# Autodesk Inventor assembly: Linear slides
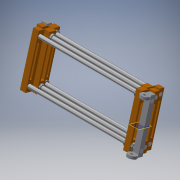
[picture p0: Inventor's stored thumbnail of the model, 180x180]
Saved by Autodesk Inventor 2019 (Build 230136000, 136)
## iProperties
Created: 2019-03-07
Part Number: Linear slides
Document SubType Name: Assembly
Designer: Delta
Mass: 697.362 g
Surface Area: 1389.66 cm^2
Volume: 258.282 cm^3
Density: 2.7 g/cm^3
Author: Delta
## Documents named in this file (6)
- C:\Robotics\2019-20_CAD\Linear Slides\Linear slides.iam
- C:\Robotics\2019-20_CAD\Linear Slides\Block_3-8.ipt
- C:\Robotics\2019-20_CAD\Linear Slides\rod_3-8_12 inch.ipt
- C:\Robotics\COTSParts\Bearings - McMaster\60595K120_FIXED ALIGNMENT  LINEAR BALL BRNG.ipt
- C:\Robotics\2019-20_CAD\Linear Slides\axil mount.ipt
- C:\Robotics\2019-20_CAD\Linear Slides\end piece.ipt
## Components (20 placed, 5 different names)
1. Block_3-8:1 — Mate:3, Mate:4, Mate:9, Mate:11, Mate:13, Mate:14, Mate:20
2. Block_3-8:2 — Mate:5, Mate:6, Mate:10, Mate:12, Mate:17, Mate:18, Mate:23, Mate:24
3. rod_3-8_12 inch:1 — Mate:4, Mate:11, Mate:27, Flush:7, Mate:49
4. rod_3-8_12 inch:2 — Mate:5, Mate:10, Flush:4, Mate:31
5. rod_3-8_12 inch:3 — Mate:3, Mate:9, Mate:28, Mate:50
6. rod_3-8_12 inch:4 — Mate:6, Mate:12, Flush:4, Mate:32, Flush:5
7. rod_3-8_12 inch:5 — Mate:25, Flush:2, Mate:30, Mate:43
8. rod_3-8_12 inch:6 — Mate:26, Mate:29, Flush:3, Flush:6, Mate:44
9. 60595K120_FIXED ALIGNMENT  LINEAR BALL BRNG:2 — Mate:13, Mate:26, Flush:1
10. 60595K120_FIXED ALIGNMENT  LINEAR BALL BRNG:4 — Mate:14, Mate:20, Mate:25, Flush:1
11. 60595K120_FIXED ALIGNMENT  LINEAR BALL BRNG:5 — Mate:17, Mate:23, Mate:28
12. 60595K120_FIXED ALIGNMENT  LINEAR BALL BRNG:6 — Mate:18, Mate:24, Mate:27
13. axil mount:1 — Mate:29, Flush:2, Flush:3, Mate:30
14. end piece:1 — Mate:31, Mate:32, Flush:5
15. Block_3-8:3 — Flush:6, Mate:43, Mate:44, Mate:45, Mate:46, Mate:47, Mate:48
16. Block_3-8:4 — Mate:39, Mate:40, Mate:41, Mate:42, Flush:7, Mate:49, Mate:50
17. 60595K120_FIXED ALIGNMENT  LINEAR BALL BRNG:7 — Mate:45, Mate:46
18. 60595K120_FIXED ALIGNMENT  LINEAR BALL BRNG:8 — Mate:47, Mate:48
19. 60595K120_FIXED ALIGNMENT  LINEAR BALL BRNG:9 — Mate:39, Mate:40
20. 60595K120_FIXED ALIGNMENT  LINEAR BALL BRNG:10 — Mate:41, Mate:42
## Relationships (42: Mate 35, Flush 7)
- Mate:3: Block_3-8:1 ↔ rod_3-8_12 inch:3
- Mate:4: Block_3-8:1 ↔ rod_3-8_12 inch:1
- Mate:5: Block_3-8:2 ↔ rod_3-8_12 inch:2
- Mate:6: Block_3-8:2 ↔ rod_3-8_12 inch:4
- Mate:9: Block_3-8:1 ↔ rod_3-8_12 inch:3
- Mate:10: Block_3-8:2 ↔ rod_3-8_12 inch:2
- Mate:11: Block_3-8:1 ↔ rod_3-8_12 inch:1
- Mate:12: Block_3-8:2 ↔ rod_3-8_12 inch:4
- Mate:13: Block_3-8:1 ↔ 60595K120_FIXED ALIGNMENT  LINEAR BALL BRNG:2
- Mate:14: Block_3-8:1 ↔ 60595K120_FIXED ALIGNMENT  LINEAR BALL BRNG:4
- Mate:17: Block_3-8:2 ↔ 60595K120_FIXED ALIGNMENT  LINEAR BALL BRNG:5
- Mate:18: Block_3-8:2 ↔ 60595K120_FIXED ALIGNMENT  LINEAR BALL BRNG:6
- Mate:20: Block_3-8:1 ↔ 60595K120_FIXED ALIGNMENT  LINEAR BALL BRNG:4
- Mate:23: Block_3-8:2 ↔ 60595K120_FIXED ALIGNMENT  LINEAR BALL BRNG:5
- Mate:24: Block_3-8:2 ↔ 60595K120_FIXED ALIGNMENT  LINEAR BALL BRNG:6
- Mate:25: rod_3-8_12 inch:5 ↔ 60595K120_FIXED ALIGNMENT  LINEAR BALL BRNG:4
- Mate:26: rod_3-8_12 inch:6 ↔ 60595K120_FIXED ALIGNMENT  LINEAR BALL BRNG:2
- Mate:27: rod_3-8_12 inch:1 ↔ 60595K120_FIXED ALIGNMENT  LINEAR BALL BRNG:6
- Mate:28: rod_3-8_12 inch:3 ↔ 60595K120_FIXED ALIGNMENT  LINEAR BALL BRNG:5
- Flush:1: 60595K120_FIXED ALIGNMENT  LINEAR BALL BRNG:2 ↔ 60595K120_FIXED ALIGNMENT  LINEAR BALL BRNG:4
- Mate:29: rod_3-8_12 inch:6 ↔ axil mount:1
- Flush:2: rod_3-8_12 inch:5 ↔ axil mount:1
- Flush:3: rod_3-8_12 inch:6 ↔ axil mount:1
- Mate:30: rod_3-8_12 inch:5 ↔ axil mount:1
- Flush:4: rod_3-8_12 inch:2 ↔ rod_3-8_12 inch:4
- Mate:31: rod_3-8_12 inch:2 ↔ end piece:1
- Mate:32: rod_3-8_12 inch:4 ↔ end piece:1
- Flush:5: rod_3-8_12 inch:4 ↔ end piece:1
- Mate:39: Block_3-8:4 ↔ 60595K120_FIXED ALIGNMENT  LINEAR BALL BRNG:9
- Mate:40: Block_3-8:4 ↔ 60595K120_FIXED ALIGNMENT  LINEAR BALL BRNG:9
- Mate:41: Block_3-8:4 ↔ 60595K120_FIXED ALIGNMENT  LINEAR BALL BRNG:10
- Mate:42: Block_3-8:4 ↔ 60595K120_FIXED ALIGNMENT  LINEAR BALL BRNG:10
- Flush:6: rod_3-8_12 inch:6 ↔ Block_3-8:3
- Mate:43: rod_3-8_12 inch:5 ↔ Block_3-8:3
- Mate:44: rod_3-8_12 inch:6 ↔ Block_3-8:3
- Mate:45: Block_3-8:3 ↔ 60595K120_FIXED ALIGNMENT  LINEAR BALL BRNG:7
- Mate:46: Block_3-8:3 ↔ 60595K120_FIXED ALIGNMENT  LINEAR BALL BRNG:7
- Mate:47: Block_3-8:3 ↔ 60595K120_FIXED ALIGNMENT  LINEAR BALL BRNG:8
- Mate:48: Block_3-8:3 ↔ 60595K120_FIXED ALIGNMENT  LINEAR BALL BRNG:8
- Flush:7: rod_3-8_12 inch:1 ↔ Block_3-8:4
- Mate:49: rod_3-8_12 inch:1 ↔ Block_3-8:4
- Mate:50: rod_3-8_12 inch:3 ↔ Block_3-8:4
